# Autodesk Inventor assembly: Tilt+Robot
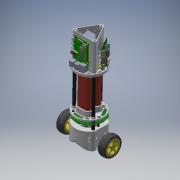
[picture p0: Inventor's stored thumbnail of the model, 180x180]
Saved by Autodesk Inventor 2018 (Build 220112000, 112)
## iProperties
Created: 2024-05-28
Part Number: Tilt+Robot
Document SubType Name: Assembly
Designer: rlndo
Sending System: Autodesk Translation Framework v13.14.0.145
Preprocessor: ST-DEVELOPER v20
Title: 36f04f60-371a-43b3-86c3-9ed645257816.stp
## Documents named in this file (3)
- C:\Users\rlndo\OneDrive\Desktop\Flamingo_model\Tilt Robot v2 2018\Tilt+Robot.iam
- C:\Users\rlndo\OneDrive\Desktop\Flamingo_model\Tilt Robot v2 2018\wheel v1.ipt
- C:\Users\rlndo\OneDrive\Desktop\Flamingo_model\Tilt Robot v2 2018\rigid_body.iam
## Components (3 placed, 2 different names)
1. wheel v1:1 — Insert:1
2. wheel v1:2 — Insert:2
3. rigid_body:1 [sub-assembly] — Insert:1, Insert:2
## Relationships (2: Insert 2)
- Insert:1: wheel v1:1 ↔ rigid_body:1
- Insert:2: wheel v1:2 ↔ rigid_body:1
